# Autodesk Inventor assembly: PeltierPower
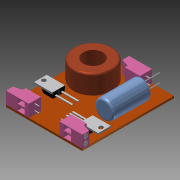
[picture p0: Inventor's stored thumbnail of the model, 180x180]
Saved by Autodesk Inventor 2014 (Build 180170000, 170)
## iProperties
Created: 2015-04-18
Part Number: PeltierPower
Document SubType Name: Assembly
Designer: Owner
Author: Owner
## Documents named in this file (7)
- C:\Users\Owner\Documents\APC\FrontEnd\IAM\Common\PeltierPower.iam
- C:\Users\Owner\Documents\APC\FrontEnd\IAM\Common\Capacitor.ipt
- C:\Users\Owner\Documents\APC\FrontEnd\IAM\Common\Diode.ipt
- C:\Users\Owner\Documents\APC\FrontEnd\IAM\Common\MOSFET.ipt
- C:\Users\Owner\Documents\APC\FrontEnd\IAM\Common\torroid.ipt
- C:\Users\Owner\Documents\APC\FrontEnd\IAM\Common\PerfBoard_Peltier.ipt
- C:\Users\Owner\Documents\APC\FrontEnd\IAM\Common\ScrewTerminal.ipt
## Components (8 placed, 6 different names)
1. Capacitor:1 — Tangent:1
2. Diode:1 — Mate:2, Flush:5
3. MOSFET:1 — Mate:3, Flush:6
4. torroid:1 — Mate:4
5. PerfBoard_Peltier:1 — Mate:2, Mate:3, Mate:4, Tangent:1, Mate:5, Flush:1, Flush:2, Mate:6, Flush:3, Flush:4, Flush:5, Flush:6, Mate:7, Flush:7
6. ScrewTerminal:1 — Mate:6, Flush:3, Flush:4
7. ScrewTerminal:2 — Mate:7, Flush:7
8. ScrewTerminal:3 — Mate:5, Flush:1, Flush:2
## Relationships (14: Flush 7, Mate 6, Tangent 1)
- Mate:2: Diode:1 ↔ PerfBoard_Peltier:1
- Mate:3: MOSFET:1 ↔ PerfBoard_Peltier:1
- Mate:4: torroid:1 ↔ PerfBoard_Peltier:1
- Tangent:1: Capacitor:1 ↔ PerfBoard_Peltier:1
- Mate:5: PerfBoard_Peltier:1 ↔ ScrewTerminal:3
- Flush:1: PerfBoard_Peltier:1 ↔ ScrewTerminal:3
- Flush:2: PerfBoard_Peltier:1 ↔ ScrewTerminal:3
- Mate:6: PerfBoard_Peltier:1 ↔ ScrewTerminal:1
- Flush:3: PerfBoard_Peltier:1 ↔ ScrewTerminal:1
- Flush:4: PerfBoard_Peltier:1 ↔ ScrewTerminal:1
- Flush:5: Diode:1 ↔ PerfBoard_Peltier:1
- Flush:6: MOSFET:1 ↔ PerfBoard_Peltier:1
- Mate:7: PerfBoard_Peltier:1 ↔ ScrewTerminal:2
- Flush:7: PerfBoard_Peltier:1 ↔ ScrewTerminal:2
